# Autodesk Inventor assembly: JAW-COUPLING-ID22MM
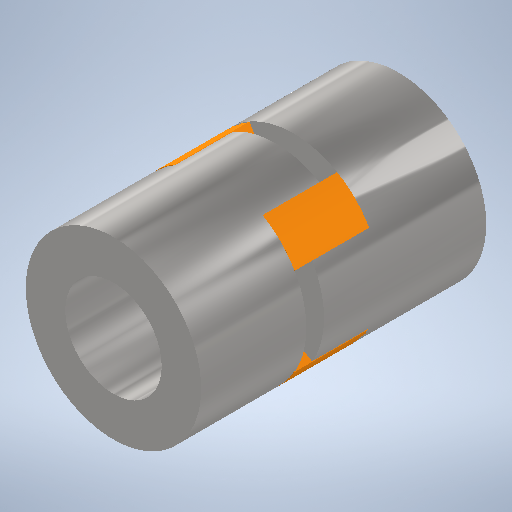
[picture p0: Inventor's stored thumbnail of the model, 512x512]
Saved by Autodesk Inventor 2025.3 (Build 293356030, 356C)
## iProperties
Created: 2025-10-06
Part Number: JAW-COUPLING-ID22MM
Document SubType Name: Assembly
Designer: lstk1ng
Author: lstk1ng
## Documents named in this file (4)
- C:\Users\lstk1ng\Documents\UPC\UPC-10\PROYECTO MECATRONICO 1\DISEÑO MECANICO\COMPONENTS\JAW-COUPLING-ID22MM.iam
- C:\Users\lstk1ng\Documents\UPC\UPC-10\PROYECTO MECATRONICO 1\DISEÑO MECANICO\COMPONENTS\NYLON-JAW.ipt
- C:\Users\lstk1ng\Documents\UPC\UPC-10\PROYECTO MECATRONICO 1\DISEÑO MECANICO\COMPONENTS\20MM JAW.ipt
- C:\Users\lstk1ng\Documents\UPC\UPC-10\PROYECTO MECATRONICO 1\DISEÑO MECANICO\COMPONENTS\22MM JAW.ipt
## Components (3 placed, 3 different names)
1. NYLON-JAW:1 — Mate:1, Mate:2, Mate:3, Mate:4, Mate:5, Mate:6
2. 20MM JAW:1 — Mate:1, Mate:2, Mate:4
3. 22MM JAW:1 — Mate:3, Mate:5, Mate:6
## Relationships (6: Mate 6)
- Mate:1: NYLON-JAW:1 ↔ 20MM JAW:1
- Mate:2: NYLON-JAW:1 ↔ 20MM JAW:1
- Mate:3: NYLON-JAW:1 ↔ 22MM JAW:1
- Mate:4: NYLON-JAW:1 ↔ 20MM JAW:1
- Mate:5: NYLON-JAW:1 ↔ 22MM JAW:1
- Mate:6: NYLON-JAW:1 ↔ 22MM JAW:1
